# Autodesk Inventor assembly: Fr.wing_cradle
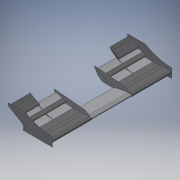
[picture p0: Inventor's stored thumbnail of the model, 180x180]
Saved by Autodesk Inventor 2018.2 (Build 222227000, 227)
## iProperties
Created: 2018-03-06
Part Number: Fr.wing_cradle
Material: 一般
Document SubType Name: Assembly
Designer: ku_sk
Author: ku_sk
## Documents named in this file (7)
- C:\Users\ku_sk\Documents\Inventor\Aero\KS-15\Fr.wing\cradle\base_model\Fr.wing_cradle\Fr.wing_cradle.iam
- C:\Users\ku_sk\Documents\Inventor\Aero\KS-15\Fr.wing\cradle\base_model\Fr.wing_cradle\bracket.ipt
- C:\Users\ku_sk\Documents\Inventor\Aero\KS-15\Fr.wing\cradle\base_model\Fr.wing_cradle\centerflap.ipt
- C:\Users\ku_sk\Documents\Inventor\Aero\KS-15\Fr.wing\cradle\base_model\Fr.wing_cradle\sideflap.ipt
- C:\Users\ku_sk\Documents\Inventor\Aero\KS-15\Fr.wing\cradle\base_model\Fr.wing_cradle\sideflap_MIR.ipt
- C:\Users\ku_sk\Documents\Inventor\Aero\KS-15\Fr.wing\cradle\base_model\Fr.wing_cradle\endplate.ipt
- C:\Users\ku_sk\Documents\Inventor\Aero\KS-15\Fr.wing\cradle\base_model\Fr.wing_cradle\endplate1.ipt
## Components (7 placed, 6 different names)
1. bracket:1 — メイト:3, メイト:5, メイト:8, メイト:9
2. centerflap:1 — フラッシュ:1, メイト:1, メイト:2, メイト:3, メイト:4, メイト:6, メイト:7, メイト:8, メイト:9, メイト:10, メイト:11
3. sideflap:1 — メイト:5, メイト:10, メイト:11, メイト:12, メイト:13, メイト:15
4. bracket:2 — メイト:2, メイト:6, メイト:7
5. sideflap_MIR:1 — メイト:4, メイト:12, メイト:13, メイト:14
6. endplate:1 — フラッシュ:2, フラッシュ:3, メイト:14, 角度:1
7. endplate1:1 — フラッシュ:2, フラッシュ:3, メイト:15
## Relationships (19: Mate 15, Flush 3, Angle 1)
- フラッシュ:1 [Flush]: centerflap:1
- メイト:1 [Mate]: centerflap:1
- メイト:2 [Mate]: centerflap:1 ↔ bracket:2
- メイト:3 [Mate]: bracket:1 ↔ centerflap:1
- メイト:4 [Mate]: centerflap:1 ↔ sideflap_MIR:1
- メイト:5 [Mate]: bracket:1 ↔ sideflap:1
- メイト:6 [Mate]: centerflap:1 ↔ bracket:2
- メイト:7 [Mate]: centerflap:1 ↔ bracket:2
- メイト:8 [Mate]: bracket:1 ↔ centerflap:1
- メイト:9 [Mate]: bracket:1 ↔ centerflap:1
- メイト:10 [Mate]: centerflap:1 ↔ sideflap:1
- メイト:11 [Mate]: centerflap:1 ↔ sideflap:1
- メイト:12 [Mate]: sideflap:1 ↔ sideflap_MIR:1
- メイト:13 [Mate]: sideflap:1 ↔ sideflap_MIR:1
- フラッシュ:2 [Flush]: endplate:1 ↔ endplate1:1
- フラッシュ:3 [Flush]: endplate:1 ↔ endplate1:1
- メイト:14 [Mate]: sideflap_MIR:1 ↔ endplate:1
- メイト:15 [Mate]: sideflap:1 ↔ endplate1:1
- 角度:1 [Angle] (0 deg): endplate:1
